# Autodesk Inventor assembly: wheel3
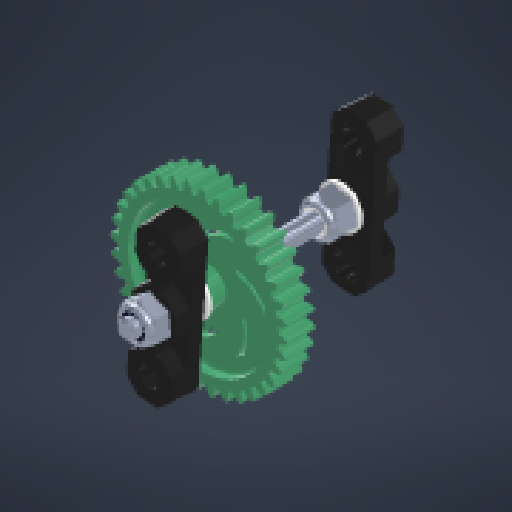
[picture p0: Inventor's stored thumbnail of the model, 512x512]
Saved by Autodesk Inventor 2024 (Build 280153000, 153)
## iProperties
Created: 2023-08-09
Part Number: wheel3
Document SubType Name: Assembly
Designer: macbook
Author: macbook
## Documents named in this file (9)
- \\Mac\Home\Desktop\code\7899V-VRC-OVER-UNDER\Cad\VEX-CAD-Inventor-1.4.0\Assembly\v0.2\wheel3.iam
- \\Mac\Home\Desktop\code\7899V-VRC-OVER-UNDER\Cad\VEX-CAD-Inventor-1.4.0\Motion\Gears\LS 36T Gear.ipt
- \\Mac\Home\Desktop\code\7899V-VRC-OVER-UNDER\Cad\VEX-CAD-Inventor-1.4.0\Motion\Shaft LS\Bearing Flat.ipt
- \\Mac\Home\Desktop\code\7899V-VRC-OVER-UNDER\Cad\VEX-CAD-Inventor-1.4.0\Motion\Spacers\Washer Teflon\TWasher .375 OD x .03125.ipt
- \\Mac\Home\Desktop\code\7899V-VRC-OVER-UNDER\Cad\VEX-CAD-Inventor-1.4.0\Motion\Spacers\Washer Teflon.ipt
- \\Mac\Home\Desktop\code\7899V-VRC-OVER-UNDER\Cad\VEX-CAD-Inventor-1.4.0\Structure\Hardware\Screw Steel - Star.ipt
- \\Mac\Home\Desktop\code\7899V-VRC-OVER-UNDER\Cad\VEX-CAD-Inventor-1.4.0\Structure\Hardware\Nut Nylock.ipt
- \\Mac\Home\Desktop\code\7899V-VRC-OVER-UNDER\Cad\VEX-CAD-Inventor-1.4.0\Structure\Hardware\Nut Thin Nylock.ipt
- \\Mac\Home\Desktop\code\7899V-VRC-OVER-UNDER\Cad\VEX-CAD-Inventor-1.4.0\Structure\Hardware\Screw Steel - Star\SScrew Star Smooth 2.250.ipt
## Components (9 placed, 6 different names)
1. LS 36T Gear:1 — Insert:11
2. TWasher .375 OD x .03125:1 — Insert:16
3. SScrew Star Smooth 2.250:3 — Insert:26
4. Nut Nylock:3 — Insert:24
5. Nut Nylock:4 — Insert:11
6. Bearing Flat:2 — Insert:16, Insert:18, Insert:27, Insert:28
7. Nut Thin Nylock:1 — Insert:18
8. Bearing Flat:4 — Insert:25, Insert:26, Insert:27, Insert:28
9. TWasher .375 OD x .03125:4 — Insert:24, Insert:25
## Relationships (9: Insert 9)
- [Insert]: LS 36T Gear:1 ↔ TWasher .375 OD x .03125:1
- Insert:11: LS 36T Gear:1 ↔ Nut Nylock:4
- Insert:16 (1.5875 mm): TWasher .375 OD x .03125:1 ↔ Bearing Flat:2
- Insert:18: Bearing Flat:2 ↔ Nut Thin Nylock:1
- Insert:24: Nut Nylock:3 ↔ TWasher .375 OD x .03125:4
- Insert:25 (1.5875 mm): Bearing Flat:4 ↔ TWasher .375 OD x .03125:4
- Insert:26: SScrew Star Smooth 2.250:3 ↔ Bearing Flat:4
- Insert:27 (38.1 mm): Bearing Flat:2 ↔ Bearing Flat:4
- Insert:28 (38.1 mm): Bearing Flat:2 ↔ Bearing Flat:4
